# Autodesk Inventor assembly: woodForkAssembly
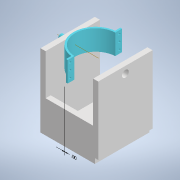
[picture p0: Inventor's stored thumbnail of the model, 180x180]
Saved by Autodesk Inventor 2021 (Build 250183000, 183)
## iProperties
Created: 2020-07-02
Part Number: woodForkAssembly
Document SubType Name: Assembly
Designer: robst
Author: robst
## Documents named in this file (6)
- C:\git\CAD-Development\robSteele\ShapeWays\TelescopeProjects\TelescopeMount\woodForkAssembly.iam
- C:\git\CAD-Development\robSteele\ShapeWays\TelescopeProjects\TelescopeMount\woodForkSupportBase.ipt
- C:\git\CAD-Development\robSteele\ShapeWays\TelescopeProjects\TelescopeMount\woodForAssemblyLeftSide.ipt
- C:\git\CAD-Development\robSteele\ShapeWays\TelescopeProjects\TelescopeMount\woodForAssemblyLeftSide_MIR.ipt
- C:\git\CAD-Development\robSteele\ShapeWays\TelescopeProjects\TelescopeMount\woodForkFrontSupport.ipt
- C:\git\CAD-Development\robSteele\ShapeWays\TelescopeProjects\TelescopeMount\tubeBracketV02.ipt
## Components (5 placed, 5 different names)
1. woodForkSupportBase:1 — Flush:1, Flush:2, Flush:3
2. woodForAssemblyLeftSide:1 — Flush:1, Insert:1
3. woodForAssemblyLeftSide_MIR:1
4. woodForkFrontSupport:1 — Flush:2, Flush:3
5. tubeBracketV02:1 — Insert:1
## Relationships (4: Flush 3, Insert 1)
- Flush:1: woodForkSupportBase:1 ↔ woodForAssemblyLeftSide:1
- Flush:2: woodForkSupportBase:1 ↔ woodForkFrontSupport:1
- Flush:3: woodForkSupportBase:1 ↔ woodForkFrontSupport:1
- Insert:1 (-25.4 mm): woodForAssemblyLeftSide:1 ↔ tubeBracketV02:1
